# Autodesk Inventor assembly: claws_endeffector_2
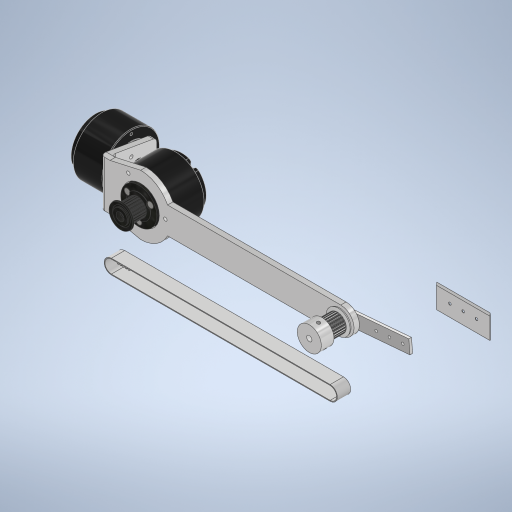
[picture p0: Inventor's stored thumbnail of the model, 512x512]
Saved by Autodesk Inventor 2024 (Build 280153000, 153)
## iProperties
Created: 2025-03-04
Part Number: claws_endeffector_2
Document SubType Name: Assembly
Designer: 1412z
Author: 1412z
## Documents named in this file (10)
- C:\Users\1412z\OneDrive\デスクトップ\rdclab\harvesting_robot\harvesting_endeffector\claws_endeffector\claws_endeffector_2.iam
- C:\Users\1412z\OneDrive\デスクトップ\rdclab\harvesting_robot\harvesting_endeffector\claws_endeffector\motor_holder\motor_holder_2.ipt
- C:\Users\1412z\OneDrive\デスクトップ\rdclab\harvesting_robot\harvesting_endeffector\claws_endeffector\GIM3505-08\GIM3505-8_with-driver.ipt
- C:\Users\1412z\OneDrive\デスクトップ\rdclab\harvesting_robot\harvesting_endeffector\claws_endeffector\misumi\HTPA22S2M100-A-V4-Z6-J3_Autodesk_Inventor_2024_20250304\HTPA22S2M100-A-V4-Z6-J3_0_a.ipt
- C:\Users\1412z\OneDrive\デスクトップ\rdclab\harvesting_robot\harvesting_endeffector\claws_endeffector\misumi\HTBN360S2M-100_Autodesk_Inventor_2024_20250304\HTBN360S2M-100_info-1-16-16.ipt
- C:\Users\1412z\OneDrive\デスクトップ\rdclab\harvesting_robot\harvesting_endeffector\claws_endeffector\misumi\SFL674ZZ_Autodesk_Inventor_2024_20250304\SFL674ZZ.ipt
- C:\Users\1412z\OneDrive\デスクトップ\rdclab\harvesting_robot\harvesting_endeffector\claws_endeffector\misumi\M2.5×4\M2.5×4.ipt
- C:\Users\1412z\OneDrive\デスクトップ\rdclab\harvesting_robot\harvesting_endeffector\claws_endeffector\misumi\HTPA22S2M100-K-P4_Autodesk_Inventor_2024_20250304\AIS2024\HTPA22S2M100-K-P4_a.ipt
- C:\Users\1412z\OneDrive\デスクトップ\rdclab\harvesting_robot\harvesting_endeffector\claws_endeffector\cutter_part\cutter_board.ipt
- C:\Users\1412z\OneDrive\デスクトップ\rdclab\harvesting_robot\harvesting_endeffector\claws_endeffector\cutter_part\cutter_XB210.ipt
## Components (13 placed, 9 different names)
1. motor_holder_2:1 — 回転:1, 回転:2, 回転:3, 回転:4, 回転:9, 回転:20
2. GIM3505-8_with-driver:1 — 回転:1, 回転:2, 回転:15, 回転:16
3. GIM3505-8_with-driver:2 — 回転:3, 回転:4
4. HTBN360S2M-100_info-1-16-16:1
5. SFL674ZZ:1 — 回転:9, 回転:14
6. HTPA22S2M100-K-P4_a:1 — 回転:14
7. HTPA22S2M100-A-V4-Z6-J3_0_a:1 — 回転:15, 回転:16, 回転:17, 回転:18, 回転:19
8. M2.5×4:1 — 回転:19
9. M2.5×4:2 — 回転:18
10. M2.5×4:3 — 回転:17
11. SFL674ZZ:2 — 回転:20, 回転:21
12. cutter_board:1 — 回転:21
13. cutter_XB210:1
## Relationships (13: RevoluteJoint 13)
- 回転:1 [RevoluteJoint]: motor_holder_2:1 ↔ GIM3505-8_with-driver:1
- 回転:2 [RevoluteJoint]: motor_holder_2:1 ↔ GIM3505-8_with-driver:1
- 回転:3 [RevoluteJoint]: motor_holder_2:1 ↔ GIM3505-8_with-driver:2
- 回転:4 [RevoluteJoint]: motor_holder_2:1 ↔ GIM3505-8_with-driver:2
- 回転:9 [RevoluteJoint]: motor_holder_2:1 ↔ SFL674ZZ:1
- 回転:14 [RevoluteJoint]: SFL674ZZ:1 ↔ HTPA22S2M100-K-P4_a:1
- 回転:15 [RevoluteJoint]: GIM3505-8_with-driver:1 ↔ HTPA22S2M100-A-V4-Z6-J3_0_a:1
- 回転:16 [RevoluteJoint]: GIM3505-8_with-driver:1 ↔ HTPA22S2M100-A-V4-Z6-J3_0_a:1
- 回転:17 [RevoluteJoint]: HTPA22S2M100-A-V4-Z6-J3_0_a:1 ↔ M2.5×4:3
- 回転:18 [RevoluteJoint]: HTPA22S2M100-A-V4-Z6-J3_0_a:1 ↔ M2.5×4:2
- 回転:19 [RevoluteJoint]: HTPA22S2M100-A-V4-Z6-J3_0_a:1 ↔ M2.5×4:1
- 回転:20 [RevoluteJoint]: motor_holder_2:1 ↔ SFL674ZZ:2
- 回転:21 [RevoluteJoint]: SFL674ZZ:2 ↔ cutter_board:1
